# Autodesk Inventor assembly: Y_Führung
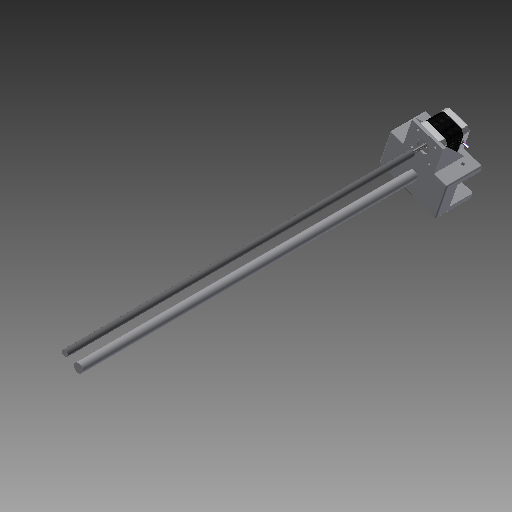
[picture p0: Inventor's stored thumbnail of the model, 512x512]
Saved by Autodesk Inventor 2019 (Build 230136000, 136)
## iProperties
Created: 2018-08-19
Part Number: Y_Führung
Document SubType Name: Assembly
Designer: Julia
Author: Julia
## Documents named in this file (5)
- C:\Users\Julia\Documents\Inventor\3d_Drucker_v04_Single_Y_Fuehrung\Y_Führung.iam
- C:\Users\Julia\Documents\Inventor\3d_Drucker_v04_Single_Y_Fuehrung\Y_Führungsstange.ipt
- C:\Users\Julia\Documents\Inventor\3d_Drucker_v04_Single_Y_Fuehrung\Y_Gewindestange.ipt
- C:\Users\Julia\Documents\Inventor\3d_Drucker_v04_Single_Y_Fuehrung\Rahmen_Y_Halterung_v2.ipt
- C:\Users\Julia\Documents\Inventor\3d_Drucker_v04_Single_Y_Fuehrung\Schrittmotor_Nema_17.ipt
## Components (4 placed, 4 different names)
1. Y_Führungsstange:1 — Mate:1, Mate:2
2. Y_Gewindestange:1 — Mate:6, Mate:7
3. Rahmen_Y_Halterung_v2:1 — Mate:1, Mate:2, Mate:3, Mate:4, Mate:5
4. Schrittmotor_Nema_17:1 — Mate:3, Mate:4, Mate:5, Mate:6, Mate:7
## Relationships (7: Mate 7)
- Mate:1: Y_Führungsstange:1 ↔ Rahmen_Y_Halterung_v2:1
- Mate:2: Y_Führungsstange:1 ↔ Rahmen_Y_Halterung_v2:1
- Mate:3: Rahmen_Y_Halterung_v2:1 ↔ Schrittmotor_Nema_17:1
- Mate:4: Rahmen_Y_Halterung_v2:1 ↔ Schrittmotor_Nema_17:1
- Mate:5: Rahmen_Y_Halterung_v2:1 ↔ Schrittmotor_Nema_17:1
- Mate:6: Y_Gewindestange:1 ↔ Schrittmotor_Nema_17:1
- Mate:7: Y_Gewindestange:1 ↔ Schrittmotor_Nema_17:1
